# Autodesk Inventor assembly: GE-11041L
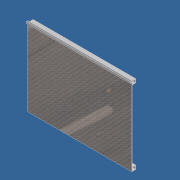
[picture p0: Inventor's stored thumbnail of the model, 180x180]
Saved by Autodesk Inventor 2012 (Build 160160000, 160)
## iProperties
Created: 2010-09-30
Part Number: GE-11041L
Document SubType Name: Assembly
Designer: mcyr
Author: mcyr
## Documents named in this file (7)
- C:\Data Folder\FRC 2012 Field\Components\GE-11041L.iam
- C:\Data Folder\FRC 2012 Field\Components\Velcro.ipt
- C:\Data Folder\FRC 2012 Field\Components\GE-11041-02.ipt
- C:\Data Folder\FRC 2012 Field\Components\GE-11041-03.ipt
- C:\Data Folder\FRC 2012 Field\Components\GE-11041-04.ipt
- C:\Data Folder\FRC 2012 Field\Components\GE-11041-01.ipt
- C:\Data Folder\FRC 2012 Field\Components\GE-11041-05.iam
## Components (7 placed, 6 different names)
1. GE-11041-02:1 — Flush:10, Mate:13, Mate:14, Flush:19
2. GE-11041-03:1 — Mate:8, Flush:13, Mate:13, Flush:19
3. GE-11041-03:2 — Mate:9, Flush:14, Flush:15, Mate:10, Mate:11, Flush:16
4. GE-11041-04:1 — Mate:6, Flush:8, Flush:9, Mate:12, Flush:17, Flush:18
5. Velcro:1 — Mate:6, Flush:8, Flush:9
6. GE-11041-01:1 — Flush:10, Mate:8, Flush:13, Mate:9, Flush:14, Flush:15, Mate:14
7. GE-11041-05:1 [sub-assembly] — Mate:10, Mate:11, Flush:16, Mate:12, Flush:17, Flush:18
## Relationships (18: Flush 10, Mate 8)
- Mate:6: GE-11041-04:1 ↔ Velcro:1
- Flush:8: GE-11041-04:1 ↔ Velcro:1
- Flush:9: GE-11041-04:1 ↔ Velcro:1
- Flush:10: GE-11041-02:1 ↔ GE-11041-01:1
- Mate:8: GE-11041-03:1 ↔ GE-11041-01:1
- Flush:13: GE-11041-03:1 ↔ GE-11041-01:1
- Mate:9: GE-11041-03:2 ↔ GE-11041-01:1
- Flush:14: GE-11041-03:2 ↔ GE-11041-01:1
- Flush:15: GE-11041-03:2 ↔ GE-11041-01:1
- Mate:10: GE-11041-03:2 ↔ GE-11041-05:1
- Mate:11: GE-11041-03:2 ↔ GE-11041-05:1
- Flush:16 (406.4 mm): GE-11041-03:2 ↔ GE-11041-05:1
- Mate:12: GE-11041-04:1 ↔ GE-11041-05:1
- Flush:17: GE-11041-04:1 ↔ GE-11041-05:1
- Flush:18: GE-11041-04:1 ↔ GE-11041-05:1
- Mate:13: GE-11041-02:1 ↔ GE-11041-03:1
- Mate:14: GE-11041-02:1 ↔ GE-11041-01:1
- Flush:19: GE-11041-02:1 ↔ GE-11041-03:1
